# Autodesk Inventor assembly: A2017_T4_07
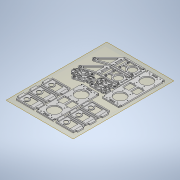
[picture p0: Inventor's stored thumbnail of the model, 180x180]
Saved by Autodesk Inventor 2020 (Build 240168000, 168)
## iProperties
Created: 2021-08-27
Part Number: A2017_T4_07
Document SubType Name: Assembly
Designer: Masato
Author: Masato
## Documents named in this file (6)
- C:\Users\naoki\Documents\Inventor\CitBrains\git_clone\SUSTAINA_ver1_0\A_T2_175\SUSTAINA-OP\Cam\A2017_T4_07.iam
- C:\Users\naoki\Documents\Inventor\CitBrains\git_clone\SUSTAINA_ver1_0\A_T2_175\SUSTAINA-OP\Cam\DisposableBoard.ipt
- C:\Users\naoki\Documents\Inventor\CitBrains\git_clone\SUSTAINA_ver1_0\A_T2_175\SUSTAINA-OP\UpperBody\Trunk\Trunk_shoulder_frame.ipt
- C:\Users\naoki\Documents\Inventor\CitBrains\git_clone\SUSTAINA_ver1_0\A_T2_175\SUSTAINA-OP\UpperBody\Trunk\Trunk_waisit_frame.ipt
- C:\Users\naoki\Documents\Inventor\CitBrains\git_clone\SUSTAINA_ver1_0\A_T2_175\SUSTAINA-OP\LowerBody\Ankle\Ankle_side_pitch_frame.ipt
- C:\Users\naoki\Documents\Inventor\CitBrains\git_clone\SUSTAINA_ver1_0\A_T2_175\SUSTAINA-OP\UpperBody\Trunk\Trunk_servo_bottom_frame.ipt
## Components (15 placed, 5 different names)
1. DisposableBoard:1 — メイト:2, メイト:1, フラッシュ:1, フラッシュ:2, メイト:4, メイト:5, メイト:6, メイト:7, メイト:8, フラッシュ:3, フラッシュ:4, メイト:15, メイト:16, メイト:20, フラッシュ:8, メイト:21, フラッシュ:9, メイト:24
2. Trunk_shoulder_frame:1 — メイト:4, メイト:10, メイト:11, 正接:1, メイト:17, メイト:18, 正接:4
3. Trunk_shoulder_frame:2 — メイト:5, フラッシュ:5, メイト:9, メイト:11
4. Trunk_waisit_frame:1 — メイト:6, フラッシュ:3, フラッシュ:4, フラッシュ:5, メイト:9, メイト:10, 正接:2, 正接:3
5. Ankle_side_pitch_frame:1 — メイト:8, メイト:14, 正接:3
6. Ankle_side_pitch_frame:2 — メイト:7, メイト:14, 正接:1, メイト:17, 正接:2, 正接:5
7. Ankle_side_pitch_frame:3 — メイト:16, メイト:19, 正接:5
8. Ankle_side_pitch_frame:4 — メイト:15, メイト:18, 正接:4, メイト:19
9. Trunk_waisit_frame:2 — フラッシュ:8, メイト:21, メイト:22, フラッシュ:10, メイト:23, フラッシュ:11
10. Trunk_servo_bottom_frame:1 — メイト:23, フラッシュ:11, メイト:24
11. Trunk_servo_bottom_frame:2 — メイト:20, フラッシュ:9, メイト:22, フラッシュ:10
12. Trunk_servo_bottom_frame:3
13. Trunk_servo_bottom_frame:4
14. Trunk_servo_bottom_frame:5
15. Trunk_servo_bottom_frame:6
## Component patterns: (3 elements, first: Trunk_servo_bottom_frame:1 + Trunk_servo_bottom_frame:2)
## Relationships (35: Mate 21, Flush 9, Tangent 5)
- メイト:2 [Mate]: DisposableBoard:1
- メイト:1 [Mate]: DisposableBoard:1
- フラッシュ:1 [Flush]: DisposableBoard:1
- フラッシュ:2 [Flush]: DisposableBoard:1
- メイト:4 [Mate]: DisposableBoard:1 ↔ Trunk_shoulder_frame:1
- メイト:5 [Mate]: DisposableBoard:1 ↔ Trunk_shoulder_frame:2
- メイト:6 [Mate]: DisposableBoard:1 ↔ Trunk_waisit_frame:1
- メイト:7 [Mate]: DisposableBoard:1 ↔ Ankle_side_pitch_frame:2
- メイト:8 [Mate]: DisposableBoard:1 ↔ Ankle_side_pitch_frame:1
- フラッシュ:3 [Flush] (2 mm): DisposableBoard:1 ↔ Trunk_waisit_frame:1
- フラッシュ:4 [Flush] (2 mm): DisposableBoard:1 ↔ Trunk_waisit_frame:1
- フラッシュ:5 [Flush]: Trunk_shoulder_frame:2 ↔ Trunk_waisit_frame:1
- メイト:9 [Mate] (2.5 mm): Trunk_shoulder_frame:2 ↔ Trunk_waisit_frame:1
- メイト:10 [Mate] (2.5 mm): Trunk_shoulder_frame:1 ↔ Trunk_waisit_frame:1
- メイト:11 [Mate] (2.5 mm): Trunk_shoulder_frame:1 ↔ Trunk_shoulder_frame:2
- メイト:14 [Mate] (2.5 mm): Ankle_side_pitch_frame:1 ↔ Ankle_side_pitch_frame:2
- 正接:1 [Tangent] (2.5 mm): Trunk_shoulder_frame:1 ↔ Ankle_side_pitch_frame:2
- メイト:15 [Mate]: DisposableBoard:1 ↔ Ankle_side_pitch_frame:4
- メイト:16 [Mate]: DisposableBoard:1 ↔ Ankle_side_pitch_frame:3
- メイト:17 [Mate] (2.5 mm): Trunk_shoulder_frame:1 ↔ Ankle_side_pitch_frame:2
- 正接:2 [Tangent] (2.5 mm): Trunk_waisit_frame:1 ↔ Ankle_side_pitch_frame:2
- 正接:3 [Tangent] (2.5 mm): Trunk_waisit_frame:1 ↔ Ankle_side_pitch_frame:1
- メイト:18 [Mate] (2.5 mm): Trunk_shoulder_frame:1 ↔ Ankle_side_pitch_frame:4
- 正接:4 [Tangent] (5 mm): Trunk_shoulder_frame:1 ↔ Ankle_side_pitch_frame:4
- メイト:19 [Mate] (2.5 mm): Ankle_side_pitch_frame:3 ↔ Ankle_side_pitch_frame:4
- 正接:5 [Tangent] (2.5 mm): Ankle_side_pitch_frame:2 ↔ Ankle_side_pitch_frame:3
- メイト:20 [Mate]: DisposableBoard:1 ↔ Trunk_servo_bottom_frame:2
- フラッシュ:8 [Flush] (2 mm): DisposableBoard:1 ↔ Trunk_waisit_frame:2
- メイト:21 [Mate]: DisposableBoard:1 ↔ Trunk_waisit_frame:2
- フラッシュ:9 [Flush] (1.5 mm): DisposableBoard:1 ↔ Trunk_servo_bottom_frame:2
- メイト:22 [Mate] (2.5 mm): Trunk_waisit_frame:2 ↔ Trunk_servo_bottom_frame:2
- フラッシュ:10 [Flush]: Trunk_waisit_frame:2 ↔ Trunk_servo_bottom_frame:2
- メイト:23 [Mate] (2.5 mm): Trunk_waisit_frame:2 ↔ Trunk_servo_bottom_frame:1
- フラッシュ:11 [Flush]: Trunk_waisit_frame:2 ↔ Trunk_servo_bottom_frame:1
- メイト:24 [Mate]: DisposableBoard:1 ↔ Trunk_servo_bottom_frame:1
